# Autodesk Inventor assembly: MeasurementChamber V3 - Assembly - Bade
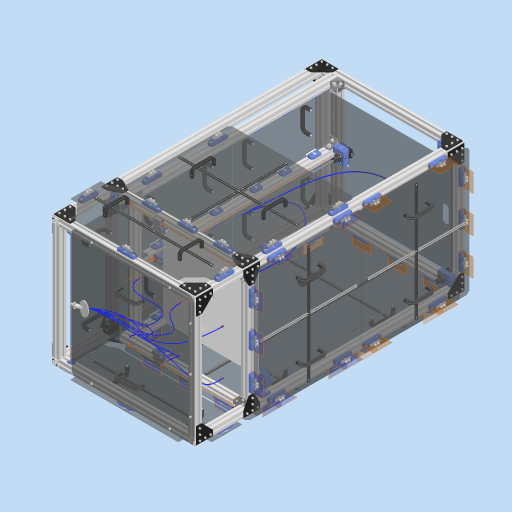
[picture p0: Inventor's stored thumbnail of the model, 512x512]
Saved by Autodesk Inventor 2023.2 (Build 272271000, 271)
## iProperties
Created: 2023-11-28
Part Number: MeasurementChamber V3 - Assembly - Bade
Document SubType Name: Assembly
Designer: Nils Bade
Author: Nils Bade
## Documents named in this file (29)
- C:\Users\nilsb\Documents\Inventor\Projektarbeit-Bade\RatRig_Bade\MeasurementChamber V3 - Assembly - Bade.iam
- C:\Users\nilsb\Documents\Inventor\Projektarbeit-Bade\RatRig_Bade\Z-Axis Transmission Assembly Back.iam
- C:\Users\nilsb\Documents\Inventor\Projektarbeit-Bade\RatRig_Bade\Z-Axis Transmission Assembly Front.iam
- C:\Users\nilsb\Documents\Inventor\Projektarbeit-Bade\RatRig_modified\Lead Screw - TR8x8-2p 1057mm Simple.ipt
- C:\Users\nilsb\Documents\Inventor\Projektarbeit-Bade\RatRig_modified\Leadscrew Constraint Front for 4040 - Assembly.iam
- C:\Users\nilsb\Documents\Inventor\Projektarbeit-Bade\RatRig_modified\Leadscrew Constraint Rear for 4040 - Assembly.iam
- C:\Users\nilsb\Documents\Inventor\Projektarbeit-Bade\RatRig_Bade\Bed Arm Back for 4040 - Assembly.iam
- C:\Users\nilsb\Documents\Inventor\Projektarbeit-Bade\RatRig_Bade\Bed Arm Left for 4040 - Assembly.iam
- C:\Users\nilsb\Documents\Inventor\Projektarbeit-Bade\RatRig_Bade\Bed Arm Right for 4040 - Assembly.iam
- C:\Users\nilsb\Documents\Inventor\Projektarbeit-Bade\RatRig_Bade\CoreXY Idler 4040 Assembly Left.iam
- C:\Users\nilsb\Documents\Inventor\Projektarbeit-Bade\RatRig_Bade\CoreXY Idler 4040 Assembly Right.iam
- C:\Users\nilsb\Documents\Inventor\Projektarbeit-Bade\Enclosure\enc-BackPanel Unten - Assembly.iam
- C:\Users\nilsb\Documents\Inventor\Projektarbeit-Bade\Enclosure\enc-BottomPanel.ipt
- C:\Users\nilsb\Documents\Inventor\Projektarbeit-Bade\RatRig_Bade\RatRig-Bade-BedAssembly.iam
- C:\Users\nilsb\Documents\Inventor\Projektarbeit-Bade\RatRig_Bade\MeasurementChamber Frame Assembly - Bade v4.iam
- MeasurementChamber Frame Assembly - Bade v4.iam
- C:\Users\nilsb\Documents\Inventor\Projektarbeit-Bade\RatRig_Bade\X-Gantry Assembly for 4040 V3.iam
- X-Gantry Assembly for 4040 V2.iam
- C:\Users\nilsb\Documents\Inventor\Projektarbeit-Bade\RatRig_Bade\CoreXY Motor Assembly Right for 4040 - V3.iam
- C:\Users\nilsb\Documents\Inventor\Projektarbeit-Bade\RatRig_Bade\CoreXY Motor Assembly Left for 4040 - V3.iam
- C:\Users\nilsb\Documents\Inventor\Projektarbeit-Bade\RatRig_Bade\HF-Kabelführung Measurement Chamber\HF-Kabelführung-V2-XGantry-Kabellängen\AIP\Kabel und Kabelbaum\HF-Kabelführung-V2-XGantry-Kabellängen.Kabelbaum1.iam
- C:\Users\nilsb\Documents\Inventor\Projektarbeit-Bade\Enclosure\enc-TopPanel V2 - Assembly no Absorber.iam
- C:\Users\nilsb\Documents\Inventor\Projektarbeit-Bade\Enclosure\enc-BackPanel Top V2 - Assembly.iam
- C:\Users\nilsb\Documents\Inventor\Projektarbeit-Bade\Enclosure\enc - FrontPanel Oben V2 - Assembly.iam
- C:\Users\nilsb\Documents\Inventor\Projektarbeit-Bade\Enclosure\enc - SidePanel Oben V2 - Assembly.iam
- C:\Users\nilsb\Documents\Inventor\Projektarbeit-Bade\Enclosure\enc-FrontPanel Unten - Assembly no Absorber.iam
- C:\Users\nilsb\Documents\Inventor\Projektarbeit-Bade\Enclosure\enc-SidePanel Unten - Assembly no Absorber.iam
- C:\Users\nilsb\Documents\Inventor\Projektarbeit-Bade\RatRig_Bade\HF-Kabelführung Measurement Chamber\HF-Kabeldurchführung-BackPanel-Multibody.ipt
- C:\Users\nilsb\Documents\Inventor\Projektarbeit-Bade\RatRig_Bade\HF-Kabelführung Measurement Chamber\HF-Kabelführung-V1-BackPlane-Kabellängen\AIP\Kabel und Kabelbaum\HF-Kabelführung-V1-BackPlane-Kabellängen.Kabelbaum1.iam
## Components (38 placed, 26 different names)
1. MeasurementChamber Frame Assembly - Bade v4:1 [sub-assembly] — Passend:69, Passend:71, Passend:100, Fluchtend:81, Fluchtend:82, Passend:102, Fluchtend:90, Fluchtend:91, Passend:112, Passend:113, Passend:114, Passend:115, Fluchtend:117, Passend:116, Passend:117, Passend:118, Passend:119, Fluchtend:118, Fluchtend:119, Passend:120, Passend:121, Passend:122, Fluchtend:120, Fluchtend:121, Passend:123, Fluchtend:122, Passend:124, Passend:125, Passend:126
2. Z-Axis Transmission Assembly Back:1 [sub-assembly] — Passend:13
3. Z-Axis Transmission Assembly Front:1 [sub-assembly] — Passend:15
4. Z-Axis Transmission Assembly Front:2 [sub-assembly] — Passend:14
5. LeadScrew - TR8x8-2p 1057mm Simple:1 — Passend:13, Passend:101
6. LeadScrew - TR8x8-2p 1057mm Simple:2 — Passend:15
7. LeadScrew - TR8x8-2p 1057mm Simple:3 — Passend:14
8. Leadscrew Constraint Front for 4040 - Assembly:1 [sub-assembly] — Fluchtend:22, Fluchtend:1
9. Leadscrew Constraint Front for 4040 - Assembly:2 [sub-assembly] — Fluchtend:22
10. Leadscrew Constraint Rear for 4040 - Assembly:1 [sub-assembly] — Fluchtend:1
11. Bed Arm Back for 4040 - Assembly:1 [sub-assembly] — Fluchtend:29
12. Bed Arm Left for 4040 - Assembly:1 [sub-assembly] — Fluchtend:24, Fluchtend:29
13. Bed Arm Right for 4040 - Assembly:1 [sub-assembly] — Fluchtend:24, Passend:78
14. CoreXY Idler 4040 Assembly Left:1 [sub-assembly]
15. CoreXY Idler 4040 Assembly Right:1 [sub-assembly]
16. CoreXY Motor Assembly Left for 4040 - V3:1 [sub-assembly]
17. CoreXY Motor Assembly Right for 4040 - V3:1 [sub-assembly]
18. enc-SidePanel Unten - Assembly no Absorber:14 [sub-assembly] — Passend:123
19. enc-SidePanel Unten - Assembly no Absorber:15 [sub-assembly] — Passend:122
20. enc-SidePanel Unten - Assembly no Absorber:16 [sub-assembly] — Fluchtend:120
21. enc-SidePanel Unten - Assembly no Absorber:17 [sub-assembly] — Fluchtend:121
22. enc-SidePanel Oben V2 - Assembly:1 [sub-assembly] — Fluchtend:117, Passend:116, Passend:117
23. enc-SidePanel Oben V2 - Assembly:2 [sub-assembly] — Passend:113, Passend:114, Passend:115
24. enc-FrontPanel Unten - Assembly no Absorber:12 [sub-assembly] — Passend:119, Passend:121, Passend:124
25. enc-FrontPanel Unten - Assembly no Absorber:13 [sub-assembly] — Fluchtend:118, Fluchtend:119, Passend:120, Fluchtend:122
26. enc-FrontPanel Oben V2 - Assembly:1 [sub-assembly] — Fluchtend:90, Fluchtend:91, Passend:112
27. enc-TopPanel V2 - Assembly no Absorber:1 [sub-assembly] — Fluchtend:81, Fluchtend:82, Passend:102
28. enc-BackPanel Top V2 - Assembly:2 [sub-assembly] — Passend:118
29. enc-BackPanel Unten - Assembly:1 [sub-assembly]
30. enc-BackPanel Unten - Assembly:2 [sub-assembly]
31. enc-BackPanel Unten - Assembly:3 [sub-assembly] — Passend:71
32. enc-BackPanel Unten - Assembly:4 [sub-assembly] — Passend:69
33. enc-BottomPanel:1
34. RatRig-Bade-BedAssembly:1 [sub-assembly] — Passend:78
35. X-Gantry Assembly for 4040 V2:2 [sub-assembly]
36. HF-Kabelführung-V2-XGantry-Kabellängen.Kabelbaum1:1 [sub-assembly] — Passend:100, Passend:101, Winkel:1, Winkel:2
37. HF-Kabeldurchführung-BackPanel-Multibody:1 — Passend:125, Passend:126, Passend:127, Passend:128
38. HF-Kabelführung-V1-BackPlane-Kabellängen.Kabelbaum1:1 [sub-assembly] — Passend:128, Fluchtend:123, Winkel:3
## Relationships (114: Mate 85, Flush 26, Angle 3)
- [Mate]: MeasurementChamber Frame Assembly - Bade v4:1 ↔ Z-Axis Transmission Assembly Back:1
- [Mate]: MeasurementChamber Frame Assembly - Bade v4:1 ↔ Z-Axis Transmission Assembly Back:1
- [Mate]: MeasurementChamber Frame Assembly - Bade v4:1 ↔ Z-Axis Transmission Assembly Back:1
- [Mate]: MeasurementChamber Frame Assembly - Bade v4:1 ↔ Z-Axis Transmission Assembly Front:1
- [Mate]: MeasurementChamber Frame Assembly - Bade v4:1 ↔ Z-Axis Transmission Assembly Front:2
- [Mate]: MeasurementChamber Frame Assembly - Bade v4:1 ↔ Z-Axis Transmission Assembly Front:2
- [Mate]: MeasurementChamber Frame Assembly - Bade v4:1 ↔ Z-Axis Transmission Assembly Front:2
- [Mate]: MeasurementChamber Frame Assembly - Bade v4:1 ↔ Z-Axis Transmission Assembly Front:1
- [Mate]: MeasurementChamber Frame Assembly - Bade v4:1 ↔ Z-Axis Transmission Assembly Front:1
- [Mate]: MeasurementChamber Frame Assembly - Bade v4:1 ↔ LeadScrew - TR8x8-2p 1057mm Simple:1
- [Mate]: MeasurementChamber Frame Assembly - Bade v4:1 ↔ LeadScrew - TR8x8-2p 1057mm Simple:2
- [Mate]: MeasurementChamber Frame Assembly - Bade v4:1 ↔ LeadScrew - TR8x8-2p 1057mm Simple:3
- Passend:13 [Mate] (-10 mm): Z-Axis Transmission Assembly Back:1 ↔ LeadScrew - TR8x8-2p 1057mm Simple:1
- Passend:14 [Mate] (-10 mm): Z-Axis Transmission Assembly Front:2 ↔ LeadScrew - TR8x8-2p 1057mm Simple:3
- Passend:15 [Mate] (-10 mm): Z-Axis Transmission Assembly Front:1 ↔ LeadScrew - TR8x8-2p 1057mm Simple:2
- [Mate]: MeasurementChamber Frame Assembly - Bade v4:1 ↔ Leadscrew Constraint Front for 4040 - Assembly:2
- [Mate]: MeasurementChamber Frame Assembly - Bade v4:1 ↔ Leadscrew Constraint Front for 4040 - Assembly:2
- [Mate] (5 mm): MeasurementChamber Frame Assembly - Bade v4:1 ↔ Leadscrew Constraint Front for 4040 - Assembly:2
- [Mate]: MeasurementChamber Frame Assembly - Bade v4:1 ↔ Leadscrew Constraint Front for 4040 - Assembly:1
- [Mate]: MeasurementChamber Frame Assembly - Bade v4:1 ↔ Leadscrew Constraint Front for 4040 - Assembly:1
- Fluchtend:22 [Flush]: Leadscrew Constraint Front for 4040 - Assembly:1 ↔ Leadscrew Constraint Front for 4040 - Assembly:2
- [Mate]: MeasurementChamber Frame Assembly - Bade v4:1 ↔ Leadscrew Constraint Rear for 4040 - Assembly:1
- [Mate]: MeasurementChamber Frame Assembly - Bade v4:1 ↔ Leadscrew Constraint Rear for 4040 - Assembly:1
- Fluchtend:1 [Flush]: Leadscrew Constraint Front for 4040 - Assembly:1 ↔ Leadscrew Constraint Rear for 4040 - Assembly:1
- [Mate]: MeasurementChamber Frame Assembly - Bade v4:1 ↔ Bed Arm Back for 4040 - Assembly:1
- [Mate]: MeasurementChamber Frame Assembly - Bade v4:1 ↔ Bed Arm Back for 4040 - Assembly:1
- [Flush]: MeasurementChamber Frame Assembly - Bade v4:1 ↔ Bed Arm Left for 4040 - Assembly:1
- [Mate]: MeasurementChamber Frame Assembly - Bade v4:1 ↔ Bed Arm Left for 4040 - Assembly:1
- [Mate]: MeasurementChamber Frame Assembly - Bade v4:1 ↔ Bed Arm Right for 4040 - Assembly:1
- [Mate]: MeasurementChamber Frame Assembly - Bade v4:1 ↔ Bed Arm Right for 4040 - Assembly:1
- Fluchtend:24 [Flush]: Bed Arm Left for 4040 - Assembly:1 ↔ Bed Arm Right for 4040 - Assembly:1
- Fluchtend:26 [Flush] (135.5 mm)
- Fluchtend:28 [Flush] (1064.95 mm)
- Fluchtend:29 [Flush]: Bed Arm Back for 4040 - Assembly:1 ↔ Bed Arm Left for 4040 - Assembly:1
- Fluchtend:30 [Flush] (1204 mm)
- Fluchtend:31 [Flush] (800 mm)
- [Mate]: MeasurementChamber Frame Assembly - Bade v4:1 ↔ enc-SidePanel Unten - Assembly no Absorber:14
- [Mate]: MeasurementChamber Frame Assembly - Bade v4:1 ↔ enc-SidePanel Unten - Assembly no Absorber:15
- [Mate] (-10 mm): MeasurementChamber Frame Assembly - Bade v4:1 ↔ enc-BackPanel Top V2 - Assembly:2
- [Mate]: MeasurementChamber Frame Assembly - Bade v4:1 ↔ enc-BackPanel Top V2 - Assembly:2
- [Mate]: MeasurementChamber Frame Assembly - Bade v4:1 ↔ enc-BackPanel Unten - Assembly:1
- [Mate]: MeasurementChamber Frame Assembly - Bade v4:1 ↔ enc-BackPanel Unten - Assembly:1
- [Mate]: MeasurementChamber Frame Assembly - Bade v4:1 ↔ enc-BackPanel Unten - Assembly:2
- [Mate]: MeasurementChamber Frame Assembly - Bade v4:1 ↔ enc-BackPanel Unten - Assembly:2
- [Mate]: MeasurementChamber Frame Assembly - Bade v4:1 ↔ enc-BackPanel Unten - Assembly:4
- Passend:69 [Mate]: MeasurementChamber Frame Assembly - Bade v4:1 ↔ enc-BackPanel Unten - Assembly:4
- [Mate]: MeasurementChamber Frame Assembly - Bade v4:1 ↔ enc-BackPanel Unten - Assembly:3
- Passend:71 [Mate]: MeasurementChamber Frame Assembly - Bade v4:1 ↔ enc-BackPanel Unten - Assembly:3
- [Mate]: MeasurementChamber Frame Assembly - Bade v4:1 ↔ enc-BackPanel Unten - Assembly:1
- [Mate]: MeasurementChamber Frame Assembly - Bade v4:1 ↔ enc-BackPanel Unten - Assembly:2
- [Mate]: MeasurementChamber Frame Assembly - Bade v4:1 ↔ enc-BackPanel Unten - Assembly:3
- [Mate]: MeasurementChamber Frame Assembly - Bade v4:1 ↔ enc-BackPanel Unten - Assembly:4
- [Mate]: MeasurementChamber Frame Assembly - Bade v4:1 ↔ enc-BottomPanel:1
- [Flush]: MeasurementChamber Frame Assembly - Bade v4:1 ↔ enc-BottomPanel:1
- [Mate]: MeasurementChamber Frame Assembly - Bade v4:1 ↔ enc-BottomPanel:1
- [Flush]: MeasurementChamber Frame Assembly - Bade v4:1 ↔ RatRig-Bade-BedAssembly:1
- Passend:78 [Mate] (18 mm): Bed Arm Right for 4040 - Assembly:1 ↔ RatRig-Bade-BedAssembly:1
- [Flush] (-327 mm): MeasurementChamber Frame Assembly - Bade v4:1 ↔ RatRig-Bade-BedAssembly:1
- [Mate]: MeasurementChamber Frame Assembly - Bade v4:1 ↔ X-Gantry Assembly for 4040 V2:2
- [Mate]: MeasurementChamber Frame Assembly - Bade v4:1 ↔ X-Gantry Assembly for 4040 V2:2
- [Mate]: MeasurementChamber Frame Assembly - Bade v4:1 ↔ X-Gantry Assembly for 4040 V2:2
- [Mate]: MeasurementChamber Frame Assembly - Bade v4:1 ↔ CoreXY Idler 4040 Assembly Right:1
- [Mate]: MeasurementChamber Frame Assembly - Bade v4:1 ↔ CoreXY Idler 4040 Assembly Left:1
- [Mate]: MeasurementChamber Frame Assembly - Bade v4:1 ↔ CoreXY Idler 4040 Assembly Left:1
- [Mate]: MeasurementChamber Frame Assembly - Bade v4:1 ↔ CoreXY Idler 4040 Assembly Left:1
- [Mate]: MeasurementChamber Frame Assembly - Bade v4:1 ↔ CoreXY Idler 4040 Assembly Right:1
- [Mate]: MeasurementChamber Frame Assembly - Bade v4:1 ↔ CoreXY Idler 4040 Assembly Right:1
- [Mate]: MeasurementChamber Frame Assembly - Bade v4:1 ↔ CoreXY Motor Assembly Left for 4040 - V3:1
- [Mate]: MeasurementChamber Frame Assembly - Bade v4:1 ↔ CoreXY Motor Assembly Left for 4040 - V3:1
- [Mate]: MeasurementChamber Frame Assembly - Bade v4:1 ↔ CoreXY Motor Assembly Left for 4040 - V3:1
- [Mate]: MeasurementChamber Frame Assembly - Bade v4:1 ↔ CoreXY Motor Assembly Right for 4040 - V3:1
- [Mate]: MeasurementChamber Frame Assembly - Bade v4:1 ↔ CoreXY Motor Assembly Right for 4040 - V3:1
- [Mate]: MeasurementChamber Frame Assembly - Bade v4:1 ↔ CoreXY Motor Assembly Right for 4040 - V3:1
- Passend:100 [Mate]: MeasurementChamber Frame Assembly - Bade v4:1 ↔ HF-Kabelführung-V2-XGantry-Kabellängen.Kabelbaum1:1
- Passend:101 [Mate]: LeadScrew - TR8x8-2p 1057mm Simple:1 ↔ HF-Kabelführung-V2-XGantry-Kabellängen.Kabelbaum1:1
- Winkel:1 [Angle] (0 deg): HF-Kabelführung-V2-XGantry-Kabellängen.Kabelbaum1:1
- Winkel:2 [Angle] (180 deg): HF-Kabelführung-V2-XGantry-Kabellängen.Kabelbaum1:1
- Fluchtend:81 [Flush]: MeasurementChamber Frame Assembly - Bade v4:1 ↔ enc-TopPanel V2 - Assembly no Absorber:1
- Fluchtend:82 [Flush]: MeasurementChamber Frame Assembly - Bade v4:1 ↔ enc-TopPanel V2 - Assembly no Absorber:1
- Passend:102 [Mate]: MeasurementChamber Frame Assembly - Bade v4:1 ↔ enc-TopPanel V2 - Assembly no Absorber:1
- Fluchtend:83 [Flush] (5 mm)
- [Flush]: MeasurementChamber Frame Assembly - Bade v4:1 ↔ enc-SidePanel Unten - Assembly no Absorber:14
- [Mate]: MeasurementChamber Frame Assembly - Bade v4:1 ↔ enc-SidePanel Unten - Assembly no Absorber:15
- [Mate]: MeasurementChamber Frame Assembly - Bade v4:1 ↔ enc-SidePanel Unten - Assembly no Absorber:17
- [Mate]: MeasurementChamber Frame Assembly - Bade v4:1 ↔ enc-SidePanel Unten - Assembly no Absorber:17
- [Flush]: MeasurementChamber Frame Assembly - Bade v4:1 ↔ enc-SidePanel Unten - Assembly no Absorber:16
- [Mate]: MeasurementChamber Frame Assembly - Bade v4:1 ↔ enc-SidePanel Unten - Assembly no Absorber:16
- Fluchtend:90 [Flush]: MeasurementChamber Frame Assembly - Bade v4:1 ↔ enc-FrontPanel Oben V2 - Assembly:1
- Fluchtend:91 [Flush]: MeasurementChamber Frame Assembly - Bade v4:1 ↔ enc-FrontPanel Oben V2 - Assembly:1
- Passend:112 [Mate]: MeasurementChamber Frame Assembly - Bade v4:1 ↔ enc-FrontPanel Oben V2 - Assembly:1
- Passend:113 [Mate]: MeasurementChamber Frame Assembly - Bade v4:1 ↔ enc-SidePanel Oben V2 - Assembly:2
- Passend:114 [Mate]: MeasurementChamber Frame Assembly - Bade v4:1 ↔ enc-SidePanel Oben V2 - Assembly:2
- Passend:115 [Mate]: MeasurementChamber Frame Assembly - Bade v4:1 ↔ enc-SidePanel Oben V2 - Assembly:2
- Fluchtend:117 [Flush]: MeasurementChamber Frame Assembly - Bade v4:1 ↔ enc-SidePanel Oben V2 - Assembly:1
- Passend:116 [Mate]: MeasurementChamber Frame Assembly - Bade v4:1 ↔ enc-SidePanel Oben V2 - Assembly:1
- Passend:117 [Mate]: MeasurementChamber Frame Assembly - Bade v4:1 ↔ enc-SidePanel Oben V2 - Assembly:1
- Passend:118 [Mate]: MeasurementChamber Frame Assembly - Bade v4:1 ↔ enc-BackPanel Top V2 - Assembly:2
- Passend:119 [Mate]: MeasurementChamber Frame Assembly - Bade v4:1 ↔ enc-FrontPanel Unten - Assembly no Absorber:12
- Fluchtend:118 [Flush]: MeasurementChamber Frame Assembly - Bade v4:1 ↔ enc-FrontPanel Unten - Assembly no Absorber:13
- Fluchtend:119 [Flush]: MeasurementChamber Frame Assembly - Bade v4:1 ↔ enc-FrontPanel Unten - Assembly no Absorber:13
- Passend:120 [Mate]: MeasurementChamber Frame Assembly - Bade v4:1 ↔ enc-FrontPanel Unten - Assembly no Absorber:13
- Passend:121 [Mate]: MeasurementChamber Frame Assembly - Bade v4:1 ↔ enc-FrontPanel Unten - Assembly no Absorber:12
- Passend:122 [Mate]: MeasurementChamber Frame Assembly - Bade v4:1 ↔ enc-SidePanel Unten - Assembly no Absorber:15
- Fluchtend:120 [Flush]: MeasurementChamber Frame Assembly - Bade v4:1 ↔ enc-SidePanel Unten - Assembly no Absorber:16
- Fluchtend:121 [Flush]: MeasurementChamber Frame Assembly - Bade v4:1 ↔ enc-SidePanel Unten - Assembly no Absorber:17
- Passend:123 [Mate]: MeasurementChamber Frame Assembly - Bade v4:1 ↔ enc-SidePanel Unten - Assembly no Absorber:14
- Fluchtend:122 [Flush]: MeasurementChamber Frame Assembly - Bade v4:1 ↔ enc-FrontPanel Unten - Assembly no Absorber:13
- Passend:124 [Mate]: MeasurementChamber Frame Assembly - Bade v4:1 ↔ enc-FrontPanel Unten - Assembly no Absorber:12
- Passend:125 [Mate]: MeasurementChamber Frame Assembly - Bade v4:1 ↔ HF-Kabeldurchführung-BackPanel-Multibody:1
- Passend:126 [Mate]: MeasurementChamber Frame Assembly - Bade v4:1 ↔ HF-Kabeldurchführung-BackPanel-Multibody:1
- Passend:127 [Mate]: HF-Kabeldurchführung-BackPanel-Multibody:1
- Passend:128 [Mate]: HF-Kabeldurchführung-BackPanel-Multibody:1 ↔ HF-Kabelführung-V1-BackPlane-Kabellängen.Kabelbaum1:1
- Fluchtend:123 [Flush]: HF-Kabelführung-V1-BackPlane-Kabellängen.Kabelbaum1:1
- Winkel:3 [Angle] (0 deg): HF-Kabelführung-V1-BackPlane-Kabellängen.Kabelbaum1:1
